# Autodesk Inventor assembly: Osnova
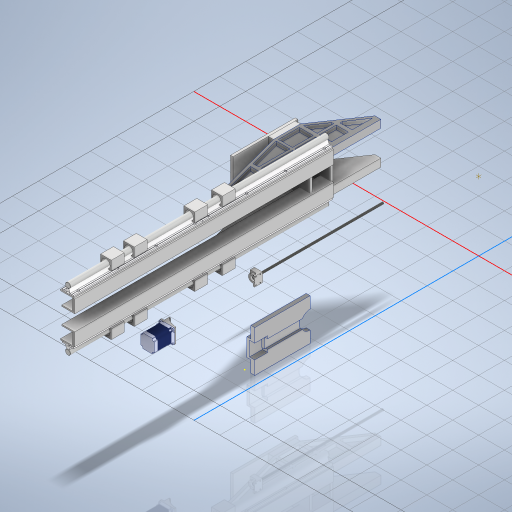
[picture p0: Inventor's stored thumbnail of the model, 512x512]
Saved by Autodesk Inventor 2024 (Build 280153000, 153)
## iProperties
Created: 2023-08-21
Part Number: Osnova
Document SubType Name: Assembly
Designer: KirikDK
Mass: 35023.4 g
Surface Area: 34965 cm^2
Volume: 16941.4 cm^3
Density: 2.06732 g/cm^3
Author: KirikDK
## Documents named in this file (16)
- C:\WorkProject\CNC_Lathe\MiniTocatka\Karkas.iam
- C:\WorkProject\CNC_Lathe\MiniTocatka\OsBase.ipt
- C:\WorkProject\CNC_Lathe\MiniTocatka\OsKrepl.ipt
- C:\WorkProject\CNC_Lathe\MiniTocatka\Vint.ipt
- C:\WorkProject\CNC_Lathe\MiniTocatka\Nozki.ipt
- C:\WorkProject\CNC_Lathe\MiniTocatka\Nozki_MIR.ipt
- C:\WorkProject\CNC_Lathe\MiniTocatka\Poperechnik.ipt
- C:\WorkProject\CNC_Lathe\MiniTocatka\NEMA-23\NEMA-23.ipt
- C:\WorkProject\CNC_Lathe\MiniTocatka\RamkaNema23.ipt
- C:\WorkProject\CNC_Lathe\MiniTocatka\650Ugol.ipt
- C:\WorkProject\CNC_Lathe\MiniTocatka\PlasticZasita.ipt
- C:\WorkProject\CNC_Lathe\MiniTocatka\MotorNatazkaOsnova.ipt
- C:\WorkProject\CNC_Lathe\MiniTocatka\MotorNatazkaPodkladka.ipt
- C:\WorkProject\CNC_Lathe\MiniTocatka\MainRailsPodsipnikKrepez.ipt
- C:\WorkProject\CNC_Lathe\MiniTocatka\LinarHC15\SBR20 Linear Rail 500 mm v7\SBR20 Linear Rail 500 mm v7.ipt
- C:\WorkProject\CNC_Lathe\MiniTocatka\SBR20_BearingBlock.ipt
## Components (30 placed, 15 different names)
1. NEMA-23:1 — Mate:82, Flush:25, Flush:26
2. RamkaNema23:1 — Mate:82, Flush:25, Flush:26
3. 650Ugol:2 — Mate:280, Flush:128, Flush:129, Mate:296, Mate:316, Mate:317, Mate:318, Flush:154
4. PlasticZasita:1
5. OsKrepl:5
6. OsBase:6 — Mate:241
7. Vint:3 — Mate:241
8. SBR20 Linear Rail 500 mm v7:7 — Mate:280, Flush:128, Flush:129, Mate:309, Mate:311, Mate:312
9. SBR20 Linear Rail 500 mm v7:8 — Mate:310
10. Poperechnik:2 — Mate:287, Flush:135
11. Nozki:4 — Mate:287, Flush:135, Flush:136, Mate:292, Mate:293, Flush:137, Mate:303, Mate:315
12. Nozki_MIR:4 — Flush:136, Flush:138, Mate:296, Mate:316
13. MotorNatazkaOsnova:2 — Mate:288
14. MotorNatazkaPodkladka:3
15. MotorNatazkaPodkladka:4 — Mate:288
16. Poperechnik:3 — Mate:292, Mate:293, Flush:137, Flush:138
17. MainRailsPodsipnikKrepez:2
18. 650Ugol:5 — Mate:303, Mate:313, Mate:314, Flush:153, Mate:315
19. SBR20 Linear Rail 500 mm v7:9
20. SBR20 Linear Rail 500 mm v7:10 — Mate:305, Mate:306, Mate:307, Mate:308
21. SBR20_BearingBlock:1 — Mate:309, Flush:148, Flush:151
22. SBR20_BearingBlock:2 — Mate:310, Flush:147, Flush:151
23. SBR20_BearingBlock:3 — Mate:311, Flush:146, Flush:152
24. SBR20_BearingBlock:4 — Mate:312, Flush:145, Flush:152
25. SBR20_BearingBlock:5 — Mate:305, Flush:148, Flush:150
26. SBR20_BearingBlock:6 — Mate:306, Flush:147, Flush:150
27. SBR20_BearingBlock:7 — Mate:307, Flush:146, Flush:149
28. SBR20_BearingBlock:8 — Mate:308, Flush:145, Flush:149
29. 650Ugol:6 — Mate:313, Mate:314, Flush:153, Flush:155
30. 650Ugol:7 — Mate:317, Mate:318, Flush:154, Flush:155
## Relationships (63: Mate 36, Flush 27)
- Mate:82: NEMA-23:1 ↔ RamkaNema23:1
- Flush:25: NEMA-23:1 ↔ RamkaNema23:1
- Flush:26: NEMA-23:1 ↔ RamkaNema23:1
- [Mate]: OsKrepl:5 ↔ OsBase:6
- [Mate]: OsKrepl:5 ↔ OsBase:6
- Mate:241: OsBase:6 ↔ Vint:3
- [Mate]: SBR20 Linear Rail 500 mm v7:7 ↔ SBR20 Linear Rail 500 mm v7:8
- [Flush]: SBR20 Linear Rail 500 mm v7:7 ↔ SBR20 Linear Rail 500 mm v7:8
- [Mate]: SBR20 Linear Rail 500 mm v7:7 ↔ SBR20 Linear Rail 500 mm v7:8
- Mate:280: 650Ugol:2 ↔ SBR20 Linear Rail 500 mm v7:7
- Flush:128: 650Ugol:2 ↔ SBR20 Linear Rail 500 mm v7:7
- Flush:129: 650Ugol:2 ↔ SBR20 Linear Rail 500 mm v7:7
- [Mate]: Poperechnik:2 ↔ Nozki_MIR:4
- [Flush]: Poperechnik:2 ↔ Nozki_MIR:4
- [Mate]: Nozki:4 ↔ MotorNatazkaPodkladka:3
- [Flush]: Nozki:4 ↔ MotorNatazkaPodkladka:3
- [Mate]: Nozki:4 ↔ MotorNatazkaPodkladka:3
- [Mate]: Nozki_MIR:4 ↔ MotorNatazkaPodkladka:4
- [Flush]: Nozki_MIR:4 ↔ MotorNatazkaPodkladka:4
- [Mate]: Nozki_MIR:4 ↔ MotorNatazkaPodkladka:4
- [Mate]: MotorNatazkaOsnova:2 ↔ MotorNatazkaPodkladka:3
- [Flush]: Nozki:4 ↔ MotorNatazkaOsnova:2
- Mate:287: Poperechnik:2 ↔ Nozki:4
- Flush:135: Poperechnik:2 ↔ Nozki:4
- Mate:288: MotorNatazkaOsnova:2 ↔ MotorNatazkaPodkladka:4
- Flush:136: Nozki:4 ↔ Nozki_MIR:4
- Mate:292: Nozki:4 ↔ Poperechnik:3
- Mate:293: Nozki:4 ↔ Poperechnik:3
- Flush:137: Nozki:4 ↔ Poperechnik:3
- Flush:138: Nozki_MIR:4 ↔ Poperechnik:3
- Mate:296: 650Ugol:2 ↔ Nozki_MIR:4
- [Mate]: SBR20 Linear Rail 500 mm v7:9 ↔ SBR20 Linear Rail 500 mm v7:10
- [Flush]: SBR20 Linear Rail 500 mm v7:9 ↔ SBR20 Linear Rail 500 mm v7:10
- [Mate]: SBR20 Linear Rail 500 mm v7:9 ↔ SBR20 Linear Rail 500 mm v7:10
- [Mate]: 650Ugol:5 ↔ SBR20 Linear Rail 500 mm v7:9
- [Flush]: 650Ugol:5 ↔ SBR20 Linear Rail 500 mm v7:9
- [Flush]: 650Ugol:5 ↔ SBR20 Linear Rail 500 mm v7:9
- Mate:303: Nozki:4 ↔ 650Ugol:5
- Mate:305: SBR20 Linear Rail 500 mm v7:10 ↔ SBR20_BearingBlock:5
- Mate:306: SBR20 Linear Rail 500 mm v7:10 ↔ SBR20_BearingBlock:6
- Mate:307: SBR20 Linear Rail 500 mm v7:10 ↔ SBR20_BearingBlock:7
- Mate:308: SBR20 Linear Rail 500 mm v7:10 ↔ SBR20_BearingBlock:8
- Mate:309: SBR20 Linear Rail 500 mm v7:7 ↔ SBR20_BearingBlock:1
- Mate:310: SBR20 Linear Rail 500 mm v7:8 ↔ SBR20_BearingBlock:2
- Mate:311: SBR20 Linear Rail 500 mm v7:7 ↔ SBR20_BearingBlock:3
- Mate:312: SBR20 Linear Rail 500 mm v7:7 ↔ SBR20_BearingBlock:4
- Flush:145: SBR20_BearingBlock:4 ↔ SBR20_BearingBlock:8
- Flush:146: SBR20_BearingBlock:3 ↔ SBR20_BearingBlock:7
- Flush:147: SBR20_BearingBlock:2 ↔ SBR20_BearingBlock:6
- Flush:148: SBR20_BearingBlock:1 ↔ SBR20_BearingBlock:5
- Flush:149: SBR20_BearingBlock:7 ↔ SBR20_BearingBlock:8
- Flush:150: SBR20_BearingBlock:5 ↔ SBR20_BearingBlock:6
- Flush:151: SBR20_BearingBlock:1 ↔ SBR20_BearingBlock:2
- Flush:152: SBR20_BearingBlock:3 ↔ SBR20_BearingBlock:4
- Mate:313: 650Ugol:5 ↔ 650Ugol:6
- Mate:314: 650Ugol:5 ↔ 650Ugol:6
- Flush:153: 650Ugol:5 ↔ 650Ugol:6
- Mate:315: Nozki:4 ↔ 650Ugol:5
- Mate:316: 650Ugol:2 ↔ Nozki_MIR:4
- Mate:317: 650Ugol:2 ↔ 650Ugol:7
- Mate:318: 650Ugol:2 ↔ 650Ugol:7
- Flush:154: 650Ugol:2 ↔ 650Ugol:7
- Flush:155: 650Ugol:6 ↔ 650Ugol:7
## Named parameters: d387_d6 = 0 mm, d388_d7 = 0 mm, d451_d446_d433_d428 = 0 mm, d452_d447_d434_d429 = 0 mm, d453_d448_d435_d430 = 0 mm, d458_d320 = 0 mm, d459_d321 = 0 mm, d460_d322 = 0 mm, d461_d323 = 0 mm, d462_d324 = 0 mm, d463_d325 = 0 mm, d464_d326 = 0 mm, d465_d327 = 0 mm, d466_d191 = 0 mm, d467_d193 = 0 mm, d487_d451_d446_d433_d428 = 0 mm, d488_d452_d447_d434_d429 = 0 mm, d489_d453_d448_d435_d430 = 0 mm, d490_d454 = 0 mm, d491_d455 = 0 mm, d492_d456 = 0 mm
